# Autodesk Inventor assembly: FronWheelDriveAssembly
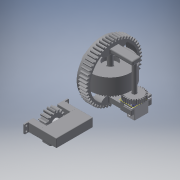
[picture p0: Inventor's stored thumbnail of the model, 180x180]
Saved by Autodesk Inventor 2018 (Build 220112000, 112)
## iProperties
Created: 2018-10-19
Part Number: FronWheelDriveAssembly
Document SubType Name: Assembly
Designer: reide
Author: reide
## Documents named in this file (11)
- C:\Users\reide\OneDrive\Documents\Inventor\TSA\2019\Animatronics\Glyptodon\Glyptodon Work\FronWheelDriveAssembly.iam
- C:\Users\reide\OneDrive\Documents\Inventor\TSA\2019\Animatronics\Glyptodon\Glyptodon Work\Front Wheel Drive\correct_wheel.ipt
- C:\Users\reide\OneDrive\Documents\Inventor\TSA\2019\Animatronics\Glyptodon\Glyptodon Work\Front Wheel Drive\wheel gear.ipt
- C:\Users\reide\OneDrive\Documents\Inventor\TSA\2019\Animatronics\Glyptodon\Glyptodon Work\Front Wheel Drive\wheelframe.ipt
- C:\Users\reide\OneDrive\Documents\Inventor\TSA\2019\Animatronics\Glyptodon\Glyptodon Work\Front Wheel Drive\wheelframe2NEW.ipt
- C:\Users\reide\OneDrive\Documents\Inventor\TSA\2019\Animatronics\Glyptodon\Mock Parts\servo (2).ipt
- C:\Users\reide\OneDrive\Documents\Inventor\TSA\2019\Animatronics\Glyptodon\Glyptodon Work\Front Wheel Drive\WheelRing.ipt
- C:\Users\reide\OneDrive\Documents\Inventor\TSA\2019\Animatronics\Glyptodon\Glyptodon Work\Front Wheel Drive\smallergear.ipt
- C:\Users\reide\OneDrive\Documents\Inventor\TSA\2019\Animatronics\Glyptodon\Glyptodon Work\Front Wheel Drive\steer_servo_mount1.ipt
- C:\Users\reide\OneDrive\Documents\Inventor\TSA\2019\Animatronics\Glyptodon\Glyptodon Work\Front Wheel Drive\steer_servo_mount2.ipt
- C:\Users\reide\OneDrive\Documents\Inventor\TSA\2019\Animatronics\Glyptodon\Glyptodon Work\Front Wheel Drive\SteerServoClamp.ipt
## Components (12 placed, 10 different names)
1. correct_wheel:1 — Mate:7, Flush:3
2. wheel gear:1 — Mate:6, Flush:3
3. wheelframe:1 — Mate:1, Flush:1, Mate:2, Mate:3, Mate:4, Flush:2, Mate:5, Mate:7, Flush:4, Flush:11
4. wheelframe2NEW:1 — Mate:1, Flush:1, Mate:2, Mate:3
5. servo (2):1 — Mate:4, Flush:2, Mate:5, Mate:6
6. WheelRing:1 — Flush:4
7. smallergear:1 — Mate:13, Mate:14
8. steer_servo_mount1:1 — Flush:5, Flush:6, Flush:7, Flush:8, Mate:8, Mate:9, Flush:9, Flush:10, Mate:10, Mate:11, Mate:12, Mate:15, Mate:16, Mate:17
9. steer_servo_mount2:1 — Flush:5, Flush:6, Flush:7, Flush:8, Mate:8
10. SteerServoClamp:1 — Mate:15, Mate:16, Mate:17
11. servo (2):2 — Mate:10, Mate:11, Mate:12, Mate:13, Mate:14
12. steer_servo_mount2:2 — Mate:9, Flush:9, Flush:10, Flush:11
## Relationships (28: Mate 17, Flush 11)
- Mate:1: wheelframe:1 ↔ wheelframe2NEW:1
- Flush:1: wheelframe:1 ↔ wheelframe2NEW:1
- Mate:2: wheelframe:1 ↔ wheelframe2NEW:1
- Mate:3: wheelframe:1 ↔ wheelframe2NEW:1
- Mate:4: wheelframe:1 ↔ servo (2):1
- Flush:2: wheelframe:1 ↔ servo (2):1
- Mate:5: wheelframe:1 ↔ servo (2):1
- Mate:6: wheel gear:1 ↔ servo (2):1
- Mate:7: correct_wheel:1 ↔ wheelframe:1
- Flush:3: correct_wheel:1 ↔ wheel gear:1
- Flush:4: wheelframe:1 ↔ WheelRing:1
- Flush:5: steer_servo_mount1:1 ↔ steer_servo_mount2:1
- Flush:6: steer_servo_mount1:1 ↔ steer_servo_mount2:1
- Flush:7: steer_servo_mount1:1 ↔ steer_servo_mount2:1
- Flush:8: steer_servo_mount1:1 ↔ steer_servo_mount2:1
- Mate:8: steer_servo_mount1:1 ↔ steer_servo_mount2:1
- Mate:9: steer_servo_mount1:1 ↔ steer_servo_mount2:2
- Flush:9: steer_servo_mount1:1 ↔ steer_servo_mount2:2
- Flush:10: steer_servo_mount1:1 ↔ steer_servo_mount2:2
- Mate:10: steer_servo_mount1:1 ↔ servo (2):2
- Mate:11: steer_servo_mount1:1 ↔ servo (2):2
- Mate:12 (0.5 mm): steer_servo_mount1:1 ↔ servo (2):2
- Mate:13: smallergear:1 ↔ servo (2):2
- Mate:14: smallergear:1 ↔ servo (2):2
- Mate:15: steer_servo_mount1:1 ↔ SteerServoClamp:1
- Mate:16: steer_servo_mount1:1 ↔ SteerServoClamp:1
- Mate:17: steer_servo_mount1:1 ↔ SteerServoClamp:1
- Flush:11: wheelframe:1 ↔ steer_servo_mount2:2
